# Autodesk Inventor assembly: SiCMonoFilamentMicroheaterPrintHead
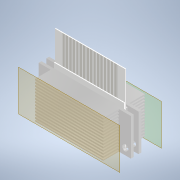
[picture p0: Inventor's stored thumbnail of the model, 180x180]
Saved by Autodesk Inventor 2021 (Build 250183000, 183)
## iProperties
Created: 2021-10-17
Part Number: SiCMonoFilamentMicroheaterPrintHead
Document SubType Name: Assembly
Designer: Unit-005
Author: Unit-005
## Documents named in this file (7)
- C:\Users\Unit-005\Documents\Inventor\SiC_Monofilament_MicroheaterPrinthead\SiCMonoFilamentMicroheaterPrintHead.iam
- C:\Users\Unit-005\Documents\Inventor\SiC_Monofilament_MicroheaterPrinthead\Al2O3PowerSideSubstrate.ipt
- C:\Users\Unit-005\Documents\Inventor\SiC_Monofilament_MicroheaterPrinthead\Leads.ipt
- C:\Users\Unit-005\Documents\Inventor\SiC_Monofilament_MicroheaterPrinthead\SiCElement.ipt
- C:\Users\Unit-005\Documents\Inventor\SiC_Monofilament_MicroheaterPrinthead\ContactPlate.ipt
- C:\Users\Unit-005\Documents\Inventor\SiC_Monofilament_MicroheaterPrinthead\ExternalHeatSinkandClamp.ipt
- C:\Users\Unit-005\Documents\Inventor\SiC_Monofilament_MicroheaterPrinthead\SiliconePad.ipt
## Components (8 placed, 6 different names)
1. Al2O3PowerSideSubstrate:1 — Mate:2, Flush:1, Mate:3, Mate:5, Mate:9, Mate:11, Flush:10
2. Leads:1 — Mate:2, Flush:1, Mate:3, Mate:4, Mate:7
3. SiCElement:1 — Mate:4, Mate:5, Flush:2, Mate:6, Mate:7, Mate:8
4. ContactPlate:1 — Flush:2, Mate:6, Mate:8, Flush:4, Flush:5, Mate:12, Flush:9
5. ExternalHeatSinkandClamp:1 — Flush:3, Flush:4, Flush:5, Flush:6, Flush:8
6. ExternalHeatSinkandClamp:2 — Mate:9, Flush:6, Mate:10, Flush:7
7. SiliconePad:1 — Mate:11, Flush:7, Flush:10
8. SiliconePad:2 — Mate:12, Flush:8, Flush:9
## Relationships (21: Mate 11, Flush 10)
- Mate:2: Al2O3PowerSideSubstrate:1 ↔ Leads:1
- Flush:1: Al2O3PowerSideSubstrate:1 ↔ Leads:1
- Mate:3: Al2O3PowerSideSubstrate:1 ↔ Leads:1
- Mate:4 (0.0675 mm): Leads:1 ↔ SiCElement:1
- Mate:5 (-0.0675 mm): Al2O3PowerSideSubstrate:1 ↔ SiCElement:1
- Flush:2 (0.0675 mm): SiCElement:1 ↔ ContactPlate:1
- Mate:6 (-0.0675 mm): SiCElement:1 ↔ ContactPlate:1
- Mate:7: Leads:1 ↔ SiCElement:1
- Mate:8: SiCElement:1 ↔ ContactPlate:1
- Flush:3: ExternalHeatSinkandClamp:1
- Flush:4 (-1.58 mm): ContactPlate:1 ↔ ExternalHeatSinkandClamp:1
- Flush:5 (1 mm): ContactPlate:1 ↔ ExternalHeatSinkandClamp:1
- Mate:9 (1.58 mm): Al2O3PowerSideSubstrate:1 ↔ ExternalHeatSinkandClamp:2
- Flush:6: ExternalHeatSinkandClamp:1 ↔ ExternalHeatSinkandClamp:2
- Mate:10: ExternalHeatSinkandClamp:2
- Mate:11: Al2O3PowerSideSubstrate:1 ↔ SiliconePad:1
- Flush:7: ExternalHeatSinkandClamp:2 ↔ SiliconePad:1
- Mate:12: ContactPlate:1 ↔ SiliconePad:2
- Flush:8: ExternalHeatSinkandClamp:1 ↔ SiliconePad:2
- Flush:9: ContactPlate:1 ↔ SiliconePad:2
- Flush:10: Al2O3PowerSideSubstrate:1 ↔ SiliconePad:1
